# Autodesk Inventor assembly: engine working
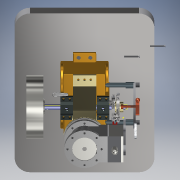
[picture p0: Inventor's stored thumbnail of the model, 180x180]
Saved by Autodesk Inventor 2017 (Build 210142000, 142)
## iProperties
Created: 2018-11-18
Part Number: engine working
Document SubType Name: Assembly
Designer: User
Author: User
## Documents named in this file (38)
- E:\Sahil's engine\engine working.iam
- E:\Sahil's engine\reverse gear base cast 2.ipt
- E:\Sahil's engine\reverse gear fly wheel.ipt
- E:\Sahil's engine\reverse gear crankshaft outer rod.ipt
- E:\Sahil's engine\reverse gear crankshaft counter weight 2.ipt
- E:\Sahil's engine\reverse gear crankshaft center rod.ipt
- E:\Sahil's engine\reverse gear  upper base bearing holder 1.ipt
- E:\Sahil's engine\reverse gear lower base bearing holder.ipt
- E:\Sahil's engine\reverse gear connecting rod 1.ipt
- E:\Sahil's engine\reverse gear bearing keeper.ipt
- E:\Sahil's engine\reverse gear crank rod 1.ipt
- E:\Sahil's engine\reverse gear crankrod pin 1.ipt
- E:\Sahil's engine\reverse gear cross head 1.ipt
- E:\Sahil's engine\reverse gear pistion rod.ipt
- E:\Sahil's engine\reverse gear piston.ipt
- E:\Sahil's engine\reverse gear stand.ipt
- C:\Users\User\Documents\Inventor\Content Center Files\R2017\en-US\AS 1427(03)\AS 1427 - M3 x 6(1).ipt
- E:\Sahil's engine\reverse gear standard 101.ipt
- E:\Sahil's engine\reverse gear lower cylinder cover.ipt
- E:\Sahil's engine\reverse gear cylinder.ipt
- E:\Sahil's engine\valvle plate.ipt
- E:\Sahil's engine\reverse gear steam chest.ipt
- E:\Sahil's engine\reverse gear steam chest cover.ipt
- E:\Sahil's engine\reverse gear lever ring stud.ipt
- E:\Sahil's engine\reverse gear eccentric 1.ipt
- E:\Sahil's engine\reverse gear lower trap.ipt
- E:\Sahil's engine\reverse gear trap holders.ipt
- E:\Sahil's engine\reverse gear essentric rod 2.ipt
- E:\Sahil's engine\reverse gear reverse lever ring.ipt
- E:\Sahil's engine\reverse gear blands.ipt
- E:\Sahil's engine\reverse gear steam chest rod valve 1.ipt
- E:\Sahil's engine\reverse gear steam chest side valve.ipt
- E:\Sahil's engine\reverse gear gear link.ipt
- E:\Sahil's engine\reverse gear rever lever.ipt
- E:\Sahil's engine\reverse gear link lever 1.ipt
- E:\Sahil's engine\reverse gear drag link.ipt
- E:\Sahil's engine\AS 1427 - M2 x 20(1).ipt
- E:\Sahil's engine\reverse gear link stud.ipt
## Components (52 placed, 37 different names)
1. reverse gear fly wheel:1 — Insert:6, Mate:2, Mate:6, Rotation:3
2. reverse gear crankshaft outer rod:1 — Insert:6, Mate:2, Mate:3, Insert:7, Mate:6, Rotation:1, Mate:51
3. reverse gear crankshaft counter weight 2:2 — Insert:4, Insert:5, Mate:41, Rotation:3
4. reverse gear crankshaft center rod:1 — Insert:4, Insert:8, Rotation:1, Mate:50
5. reverse gear crankshaft outer rod:2 — Insert:5, Mate:3, Insert:22, Insert:23, Mate:41
6. reverse gear  upper base bearing holder 1:1 — Mate:4, Flush:1, Flush:2, Flush:3, Flush:4
7. reverse gear lower base bearing holder:1 — Mate:4, Flush:1, Flush:2, Insert:7, Mate:5
8. reverse gear base cast 2:1 — Mate:5, Flush:3, Flush:4, Mate:9, Flush:7, Flush:8, Flush:15, Flush:16, Mate:13, Insert:13, Insert:14, Insert:15, Insert:16, Mate:14, Flush:17, Flush:18, Insert:20, Insert:21, Mate:53
9. reverse gear  upper base bearing holder 1:2 — Mate:8, Flush:5, Flush:6, Flush:8
10. reverse gear lower base bearing holder:2 — Mate:8, Flush:5, Flush:6, Mate:9, Flush:7
11. reverse gear connecting rod 1:1 — Mate:10, Flush:9, Flush:10, Insert:8, Mate:45, Mate:46, Mate:47, Mate:52
12. reverse gear connecting rod 1:2 — Mate:10, Flush:9, Flush:10, Mate:11, Flush:11, Flush:12
13. reverse gear bearing keeper:1 — Mate:11, Flush:11, Flush:12
14. reverse gear crankrod pin 1:1 — Mate:61, Mate:62
15. reverse gear cross head 1:1 — Mate:57, Mate:59, Mate:60
16. reverse gear pistion rod:1 — Mate:54, Mate:55, Mate:56, Mate:57
17. reverse gear piston:1 — Angle:2, Mate:54, Mate:55, Flush:30
18. reverse gear stand:1 — Flush:15, Flush:16, Mate:13, Angle:1, Angle:2
19. AS 1427 - Metric M3 x 6:1 — Insert:14
20. AS 1427 - Metric M3 x 6:2 — Insert:16
21. AS 1427 - Metric M3 x 6:3 — Insert:15
22. AS 1427 - Metric M3 x 6:4 — Insert:13
23. reverse gear standard 101:1 — Mate:14, Flush:17, Flush:18, Insert:18, Mate:56
24. reverse gear lower cylinder cover:1 — Insert:18, Insert:19, Mate:32, Mate:33, Mate:34
25. reverse gear cylinder:1 — Insert:19, Mate:15, Flush:19, Flush:20, Flush:21, Flush:22, Mate:32, Mate:33, Mate:34
26. valvle plate:1 — Mate:15, Flush:19, Flush:20, Mate:16
27. reverse gear steam chest:1 — Mate:16, Flush:21, Flush:22, Mate:17, Flush:23, Flush:24, Insert:29, Mate:69, Mate:70
28. reverse gear steam chest cover:1 — Mate:17, Flush:23, Flush:24, Angle:1, Mate:63, Mate:64, Mate:65
29. reverse gear lever ring stud:1 — Insert:20, Mate:39
30. reverse gear lever ring stud:2 — Insert:21, Mate:29
31. reverse gear eccentric 1:1 — Insert:22, Insert:24
32. reverse gear eccentric 1:2 — Insert:23, Insert:25
33. reverse gear lower trap:1 — Mate:20, Mate:21, Flush:26
34. reverse gear lower trap:2 — Mate:18, Mate:19, Flush:25
35. reverse gear trap holders:1 — Insert:24, Mate:18, Mate:19, Flush:25, Insert:27
36. reverse gear trap holders:2 — Insert:25, Mate:20, Mate:21, Flush:26, Insert:26
37. reverse gear essentric rod 2:1 — Insert:27
38. reverse gear essentric rod 2:2 — Insert:26
39. reverse gear reverse lever ring:1 — Mate:29, Mate:39, Mate:40, Mate:67, Mate:68
40. reverse gear blands:1 — Insert:29
41. reverse gear steam chest rod valve 1:1 — Mate:70, Mate:71, Mate:72
42. reverse gear steam chest side valve:1 — Mate:69, Mate:71, Mate:72
43. reverse gear gear link:1 — Mate:63, Mate:64, Mate:65, Tangent:1, Mate:66
44. reverse gear rever lever:1 — Mate:37, Mate:38, Mate:40
45. reverse gear link lever 1:1
46. reverse gear drag link:1 — Mate:37, Mate:38
47. AS 1427 - Metric M2 x 20:1
48. AS 1427 - Metric M2 x 20:2
49. reverse gear crank rod 1:1 — Mate:45, Mate:46, Mate:47, Mate:59, Mate:61, Mate:62
50. reverse gear crankshaft counter weight 2:3 — Mate:50, Mate:51, Mate:52, Mate:53
51. reverse gear link stud:1 — Tangent:1, Mate:66, Tangent:2
52. reverse gear rever lever:2 — Mate:67, Mate:68, Tangent:2
## Relationships (103: Mate 52, Flush 25, Insert 20, RelateRotation 2, Angle 2, Tangent 2)
- Insert:4: reverse gear crankshaft counter weight 2:2 ↔ reverse gear crankshaft center rod:1
- Insert:5 (-4 mm): reverse gear crankshaft counter weight 2:2 ↔ reverse gear crankshaft outer rod:2
- Insert:6: reverse gear fly wheel:1 ↔ reverse gear crankshaft outer rod:1
- Mate:2: reverse gear fly wheel:1 ↔ reverse gear crankshaft outer rod:1
- Mate:3: reverse gear crankshaft outer rod:1 ↔ reverse gear crankshaft outer rod:2
- Mate:4: reverse gear  upper base bearing holder 1:1 ↔ reverse gear lower base bearing holder:1
- Flush:1: reverse gear  upper base bearing holder 1:1 ↔ reverse gear lower base bearing holder:1
- Flush:2 (7 mm): reverse gear  upper base bearing holder 1:1 ↔ reverse gear lower base bearing holder:1
- Insert:7 (-15 mm): reverse gear crankshaft outer rod:1 ↔ reverse gear lower base bearing holder:1
- Mate:5: reverse gear lower base bearing holder:1 ↔ reverse gear base cast 2:1
- Flush:3 (29 mm): reverse gear  upper base bearing holder 1:1 ↔ reverse gear base cast 2:1
- Flush:4: reverse gear  upper base bearing holder 1:1 ↔ reverse gear base cast 2:1
- Mate:6: reverse gear fly wheel:1 ↔ reverse gear crankshaft outer rod:1
- Mate:8: reverse gear  upper base bearing holder 1:2 ↔ reverse gear lower base bearing holder:2
- Flush:5 (7 mm): reverse gear  upper base bearing holder 1:2 ↔ reverse gear lower base bearing holder:2
- Flush:6: reverse gear  upper base bearing holder 1:2 ↔ reverse gear lower base bearing holder:2
- Mate:9: reverse gear base cast 2:1 ↔ reverse gear lower base bearing holder:2
- Flush:7: reverse gear base cast 2:1 ↔ reverse gear lower base bearing holder:2
- Flush:8 (29 mm): reverse gear base cast 2:1 ↔ reverse gear  upper base bearing holder 1:2
- Mate:10: reverse gear connecting rod 1:1 ↔ reverse gear connecting rod 1:2
- Flush:9: reverse gear connecting rod 1:1 ↔ reverse gear connecting rod 1:2
- Flush:10: reverse gear connecting rod 1:1 ↔ reverse gear connecting rod 1:2
- Mate:11: reverse gear connecting rod 1:2 ↔ reverse gear bearing keeper:1
- Flush:11: reverse gear connecting rod 1:2 ↔ reverse gear bearing keeper:1
- Flush:12: reverse gear connecting rod 1:2 ↔ reverse gear bearing keeper:1
- Insert:8 (5.5 mm): reverse gear crankshaft center rod:1 ↔ reverse gear connecting rod 1:1
- Flush:15 (-58 mm): reverse gear base cast 2:1 ↔ reverse gear stand:1
- Flush:16 (53 mm): reverse gear base cast 2:1 ↔ reverse gear stand:1
- Mate:13: reverse gear base cast 2:1 ↔ reverse gear stand:1
- Insert:13 (-5.5 mm): reverse gear base cast 2:1 ↔ AS 1427 - Metric M3 x 6:4
- Insert:14 (-5.5 mm): reverse gear base cast 2:1 ↔ AS 1427 - Metric M3 x 6:1
- Insert:15 (-5.5 mm): reverse gear base cast 2:1 ↔ AS 1427 - Metric M3 x 6:3
- Insert:16 (-5.5 mm): reverse gear base cast 2:1 ↔ AS 1427 - Metric M3 x 6:2
- Mate:14: reverse gear base cast 2:1 ↔ reverse gear standard 101:1
- Flush:17: reverse gear base cast 2:1 ↔ reverse gear standard 101:1
- Flush:18 (12 mm): reverse gear base cast 2:1 ↔ reverse gear standard 101:1
- Insert:18 (-6.5 mm): reverse gear standard 101:1 ↔ reverse gear lower cylinder cover:1
- Insert:19: reverse gear lower cylinder cover:1 ↔ reverse gear cylinder:1
- Mate:15: reverse gear cylinder:1 ↔ valvle plate:1
- Flush:19: reverse gear cylinder:1 ↔ valvle plate:1
- Flush:20: reverse gear cylinder:1 ↔ valvle plate:1
- Mate:16: valvle plate:1 ↔ reverse gear steam chest:1
- Flush:21: reverse gear cylinder:1 ↔ reverse gear steam chest:1
- Flush:22: reverse gear cylinder:1 ↔ reverse gear steam chest:1
- Mate:17: reverse gear steam chest:1 ↔ reverse gear steam chest cover:1
- Flush:23: reverse gear steam chest:1 ↔ reverse gear steam chest cover:1
- Flush:24: reverse gear steam chest:1 ↔ reverse gear steam chest cover:1
- Insert:20 (-4.8 mm): reverse gear base cast 2:1 ↔ reverse gear lever ring stud:1
- Insert:21 (-4.8 mm): reverse gear base cast 2:1 ↔ reverse gear lever ring stud:2
- Insert:22 (-18 mm): reverse gear crankshaft outer rod:2 ↔ reverse gear eccentric 1:1
- Insert:23 (-12 mm): reverse gear crankshaft outer rod:2 ↔ reverse gear eccentric 1:2
- Insert:24: reverse gear eccentric 1:1 ↔ reverse gear trap holders:1
- Mate:18: reverse gear lower trap:2 ↔ reverse gear trap holders:1
- Mate:19: reverse gear lower trap:2 ↔ reverse gear trap holders:1
- Flush:25: reverse gear lower trap:2 ↔ reverse gear trap holders:1
- Insert:25: reverse gear eccentric 1:2 ↔ reverse gear trap holders:2
- Mate:20: reverse gear lower trap:1 ↔ reverse gear trap holders:2
- Mate:21: reverse gear lower trap:1 ↔ reverse gear trap holders:2
- Flush:26: reverse gear lower trap:1 ↔ reverse gear trap holders:2
- Insert:26 (-3.7 mm): reverse gear trap holders:2 ↔ reverse gear essentric rod 2:2
- Insert:27 (-3.7 mm): reverse gear trap holders:1 ↔ reverse gear essentric rod 2:1
- Rotation:1 [RelateRotation] (1 ul): reverse gear crankshaft outer rod:1 ↔ reverse gear crankshaft center rod:1
- Insert:29 (-8 mm): reverse gear steam chest:1 ↔ reverse gear blands:1
- Mate:29: reverse gear lever ring stud:2 ↔ reverse gear reverse lever ring:1
- Mate:32: reverse gear lower cylinder cover:1 ↔ reverse gear cylinder:1
- Mate:33: reverse gear lower cylinder cover:1 ↔ reverse gear cylinder:1
- Mate:34: reverse gear lower cylinder cover:1 ↔ reverse gear cylinder:1
- Angle:1 (0 deg): reverse gear stand:1 ↔ reverse gear steam chest cover:1
- Mate:37: reverse gear rever lever:1 ↔ reverse gear drag link:1
- Mate:38: reverse gear rever lever:1 ↔ reverse gear drag link:1
- Mate:39: reverse gear lever ring stud:1 ↔ reverse gear reverse lever ring:1
- Mate:40: reverse gear reverse lever ring:1 ↔ reverse gear rever lever:1
- Mate:41: reverse gear crankshaft counter weight 2:2 ↔ reverse gear crankshaft outer rod:2
- Angle:2 (0 deg): reverse gear piston:1 ↔ reverse gear stand:1
- Mate:45: reverse gear connecting rod 1:1 ↔ reverse gear crank rod 1:1
- Mate:46: reverse gear connecting rod 1:1 ↔ reverse gear crank rod 1:1
- Mate:47: reverse gear connecting rod 1:1 ↔ reverse gear crank rod 1:1
- Mate:50: reverse gear crankshaft center rod:1 ↔ reverse gear crankshaft counter weight 2:3
- Mate:51: reverse gear crankshaft outer rod:1 ↔ reverse gear crankshaft counter weight 2:3
- Mate:52: reverse gear connecting rod 1:1 ↔ reverse gear crankshaft counter weight 2:3
- Mate:53 (2.25 mm): reverse gear base cast 2:1 ↔ reverse gear crankshaft counter weight 2:3
- Mate:54: reverse gear pistion rod:1 ↔ reverse gear piston:1
- Mate:55: reverse gear pistion rod:1 ↔ reverse gear piston:1
- Mate:56: reverse gear pistion rod:1 ↔ reverse gear standard 101:1
- Mate:57: reverse gear cross head 1:1 ↔ reverse gear pistion rod:1
- Mate:59: reverse gear cross head 1:1 ↔ reverse gear crank rod 1:1
- Flush:30 (45 mm): reverse gear piston:1
- Mate:60: reverse gear cross head 1:1
- Mate:61: reverse gear crankrod pin 1:1 ↔ reverse gear crank rod 1:1
- Mate:62: reverse gear crankrod pin 1:1 ↔ reverse gear crank rod 1:1
- Rotation:3 [RelateRotation] (2.05 ul): reverse gear fly wheel:1 ↔ reverse gear crankshaft counter weight 2:2
- Mate:63: reverse gear steam chest cover:1 ↔ reverse gear gear link:1
- Mate:64: reverse gear steam chest cover:1 ↔ reverse gear gear link:1
- Mate:65: reverse gear steam chest cover:1 ↔ reverse gear gear link:1
- Tangent:1: reverse gear gear link:1 ↔ reverse gear link stud:1
- Mate:66: reverse gear gear link:1 ↔ reverse gear link stud:1
- Mate:67: reverse gear reverse lever ring:1 ↔ reverse gear rever lever:2
- Mate:68: reverse gear reverse lever ring:1 ↔ reverse gear rever lever:2
- Tangent:2: reverse gear link stud:1 ↔ reverse gear rever lever:2
- Mate:69: reverse gear steam chest:1 ↔ reverse gear steam chest side valve:1
- Mate:70: reverse gear steam chest:1 ↔ reverse gear steam chest rod valve 1:1
- Mate:71: reverse gear steam chest rod valve 1:1 ↔ reverse gear steam chest side valve:1
- Mate:72: reverse gear steam chest rod valve 1:1 ↔ reverse gear steam chest side valve:1
